# Autodesk Inventor assembly: A2017_T3_02
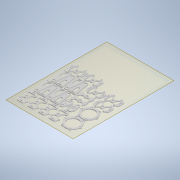
[picture p0: Inventor's stored thumbnail of the model, 180x180]
Saved by Autodesk Inventor 2020 (Build 240168000, 168)
## iProperties
Created: 2021-08-27
Part Number: A2017_T3_02
Document SubType Name: Assembly
Designer: Masato
Author: Masato
## Documents named in this file (7)
- D:\GitHub\inventor\SUSTAINA-OP\Cam\A2017_T3_02.iam
- D:\GitHub\inventor\SUSTAINA-OP\Cam\DisposableBoard.ipt
- D:\GitHub\inventor\SUSTAINA-OP\LowerBody\Leg_joint\Leg_joint_roll_frame.ipt
- D:\GitHub\inventor\SUSTAINA-OP\LowerBody\Leg_joint\Leg_joint_slider_frame.ipt
- D:\GitHub\inventor\SUSTAINA-OP\LowerBody\Slider_crank\Slider_crank_horn.ipt
- D:\GitHub\inventor\SUSTAINA-OP\LowerBody\Ankle\Ankle_front_frame.ipt
- D:\GitHub\inventor\SUSTAINA-OP\UpperBody\Trunk\CrossRollerBearing\Outer_flange.ipt
## Components (25 placed, 6 different names)
1. DisposableBoard:1 — メイト:2, メイト:1, フラッシュ:1, フラッシュ:2, フラッシュ:12, 正接:1, フラッシュ:13, 角度:1, メイト:8, 正接:8, 角度:2, メイト:10, メイト:12, メイト:13, 角度:3, メイト:14, メイト:17
2. Outer_flange:1 — フラッシュ:7
3. Slider_crank_horn:2 — フラッシュ:4, フラッシュ:9, メイト:6, 正接:4, メイト:7, 正接:9
4. Slider_crank_horn:1 — フラッシュ:3, メイト:6, 正接:5
5. Leg_joint_roll_frame:6 — メイト:12, メイト:16, 正接:11
6. Leg_joint_roll_frame:8 — メイト:13, メイト:17, 正接:12, メイト:18
7. Leg_joint_roll_frame:10 — メイト:14, メイト:18, 正接:13
8. Leg_joint_roll_frame:1 — フラッシュ:3, フラッシュ:4, フラッシュ:5, フラッシュ:10, フラッシュ:12, 正接:1, 正接:2, メイト:8
9. Leg_joint_roll_frame:3
10. Leg_joint_roll_frame:4
11. Leg_joint_roll_frame:5 — 正接:4, 正接:5, 正接:7
12. Leg_joint_slider_frame:1 — フラッシュ:6, フラッシュ:7, フラッシュ:13, 正接:2, メイト:5, 正接:3
13. Leg_joint_slider_frame:2 — フラッシュ:5, フラッシュ:6, メイト:5, 正接:3
14. Leg_joint_slider_frame:3 — 正接:12
15. Leg_joint_slider_frame:4
16. Leg_joint_slider_frame:5
17. Leg_joint_slider_frame:6 — メイト:7
18. Leg_joint_slider_frame:7 — 正接:13
19. Leg_joint_slider_frame:8 — メイト:9
20. Outer_flange:2 — フラッシュ:9, 角度:1, 正接:7, 正接:8
21. Outer_flange:3 — 正接:10
22. Ankle_front_frame:1 — フラッシュ:10, 角度:2, 正接:9
23. Ankle_front_frame:2 — メイト:9, メイト:15, 正接:11
24. Leg_joint_roll_frame:7 — メイト:10, 角度:3, メイト:15, 正接:10
25. Leg_joint_roll_frame:11 — メイト:16
## Component patterns: (4 elements, first: Leg_joint_roll_frame:1), (4 elements, first: Leg_joint_slider_frame:1 + Leg_joint_slider_frame:2), (2 elements, first: Outer_flange:2), (2 elements, first: Ankle_front_frame:1), (2 elements, first: Leg_joint_roll_frame:7)
## Relationships (41: Mate 15, Tangent 12, Flush 11, Angle 3)
- メイト:2 [Mate]: DisposableBoard:1
- メイト:1 [Mate]: DisposableBoard:1
- フラッシュ:1 [Flush]: DisposableBoard:1
- フラッシュ:2 [Flush]: DisposableBoard:1
- フラッシュ:3 [Flush]: Slider_crank_horn:1 ↔ Leg_joint_roll_frame:1
- フラッシュ:4 [Flush]: Slider_crank_horn:2 ↔ Leg_joint_roll_frame:1
- フラッシュ:5 [Flush]: Leg_joint_roll_frame:1 ↔ Leg_joint_slider_frame:2
- フラッシュ:6 [Flush]: Leg_joint_slider_frame:1 ↔ Leg_joint_slider_frame:2
- フラッシュ:7 [Flush]: Outer_flange:1 ↔ Leg_joint_slider_frame:1
- フラッシュ:9 [Flush]: Slider_crank_horn:2 ↔ Outer_flange:2
- フラッシュ:10 [Flush]: Leg_joint_roll_frame:1 ↔ Ankle_front_frame:1
- フラッシュ:12 [Flush] (2 mm): DisposableBoard:1 ↔ Leg_joint_roll_frame:1
- 正接:1 [Tangent] (2 mm): DisposableBoard:1 ↔ Leg_joint_roll_frame:1
- フラッシュ:13 [Flush] (2 mm): DisposableBoard:1 ↔ Leg_joint_slider_frame:1
- 正接:2 [Tangent] (2.5 mm): Leg_joint_roll_frame:1 ↔ Leg_joint_slider_frame:1
- メイト:5 [Mate] (2.5 mm): Leg_joint_slider_frame:1 ↔ Leg_joint_slider_frame:2
- 正接:3 [Tangent]: Leg_joint_slider_frame:1 ↔ Leg_joint_slider_frame:2
- メイト:6 [Mate] (2.5 mm): Slider_crank_horn:2 ↔ Slider_crank_horn:1
- 正接:4 [Tangent] (2.5 mm): Slider_crank_horn:2 ↔ Leg_joint_roll_frame:5
- 正接:5 [Tangent] (2.5 mm): Slider_crank_horn:1 ↔ Leg_joint_roll_frame:5
- メイト:7 [Mate] (2.5 mm): Slider_crank_horn:2 ↔ Leg_joint_slider_frame:6
- 角度:1 [Angle] (30 deg): DisposableBoard:1 ↔ Outer_flange:2
- メイト:8 [Mate]: DisposableBoard:1 ↔ Leg_joint_roll_frame:1
- 正接:7 [Tangent] (1 mm): Leg_joint_roll_frame:5 ↔ Outer_flange:2
- 正接:8 [Tangent] (2 mm): DisposableBoard:1 ↔ Outer_flange:2
- 角度:2 [Angle] (0 deg): DisposableBoard:1 ↔ Ankle_front_frame:1
- メイト:9 [Mate] (2.5 mm): Leg_joint_slider_frame:8 ↔ Ankle_front_frame:2
- 正接:9 [Tangent] (2.5 mm): Slider_crank_horn:2 ↔ Ankle_front_frame:1
- メイト:10 [Mate]: DisposableBoard:1 ↔ Leg_joint_roll_frame:7
- メイト:12 [Mate]: DisposableBoard:1 ↔ Leg_joint_roll_frame:6
- メイト:13 [Mate]: DisposableBoard:1 ↔ Leg_joint_roll_frame:8
- 角度:3 [Angle] (-90 deg): DisposableBoard:1 ↔ Leg_joint_roll_frame:7
- メイト:14 [Mate]: DisposableBoard:1 ↔ Leg_joint_roll_frame:10
- メイト:15 [Mate] (9 mm): Ankle_front_frame:2 ↔ Leg_joint_roll_frame:7
- 正接:10 [Tangent] (4 mm): Outer_flange:3 ↔ Leg_joint_roll_frame:7
- メイト:16 [Mate] (2.5 mm): Leg_joint_roll_frame:6 ↔ Leg_joint_roll_frame:11
- 正接:11 [Tangent] (2.5 mm): Leg_joint_roll_frame:6 ↔ Ankle_front_frame:2
- メイト:17 [Mate] (2 mm): DisposableBoard:1 ↔ Leg_joint_roll_frame:8
- 正接:12 [Tangent] (2.5 mm): Leg_joint_roll_frame:8 ↔ Leg_joint_slider_frame:3
- メイト:18 [Mate] (2.5 mm): Leg_joint_roll_frame:8 ↔ Leg_joint_roll_frame:10
- 正接:13 [Tangent] (2.5 mm): Leg_joint_roll_frame:10 ↔ Leg_joint_slider_frame:7
